# Autodesk Inventor assembly: partsassembeled2
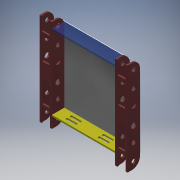
[picture p0: Inventor's stored thumbnail of the model, 180x180]
Saved by Autodesk Inventor 2017 (Build 210142000, 142)
## iProperties
Created: 2016-09-25
Part Number: partsassembeled2
Document SubType Name: Assembly
Designer: vslabsal
Author: vslabsal
## Documents named in this file (5)
- C:\Users\vslabsal\Desktop\partsassembeled2.iam
- C:\Users\vslabsal\Downloads\BK-BKT120-BasePlate-Short.ipt
- C:\Users\vslabsal\Downloads\BT-BTK120-DriveFrameTube-Rounded.ipt
- C:\Users\vslabsal\Downloads\BK-BKT120-Front.ipt
- C:\Users\vslabsal\Downloads\BK-BK120-Back.ipt
## Components (5 placed, 4 different names)
1. BK-BKT120-BasePlate-Short:1 — Rigid:1, Rigid:2, Rigid:3, Rigid:4
2. BT-BTK120-DriveFrameTube-Rounded:1 — Rigid:1
3. BT-BTK120-DriveFrameTube-Rounded:2 — Rigid:2
4. BK-BKT120-Front:1 — Rigid:3
5. BK-BK120-Back:1 — Rigid:4
## Relationships (4: WeldJoint 4)
- Rigid:1 [WeldJoint]: BK-BKT120-BasePlate-Short:1 ↔ BT-BTK120-DriveFrameTube-Rounded:1
- Rigid:2 [WeldJoint]: BK-BKT120-BasePlate-Short:1 ↔ BT-BTK120-DriveFrameTube-Rounded:2
- Rigid:3 [WeldJoint]: BK-BKT120-BasePlate-Short:1 ↔ BK-BKT120-Front:1
- Rigid:4 [WeldJoint]: BK-BKT120-BasePlate-Short:1 ↔ BK-BK120-Back:1
